# Autodesk Inventor assembly: engine working 1
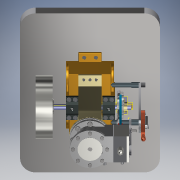
[picture p0: Inventor's stored thumbnail of the model, 180x180]
Saved by Autodesk Inventor 2017 (Build 210142000, 142)
## iProperties
Created: 2018-11-18
Part Number: engine working 1
Document SubType Name: Assembly
Designer: User
Author: User
## Documents named in this file (45)
- E:\Sahil's engine\engine working 1.iam
- E:\Sahil's engine\reverse gear base cast 2.ipt
- E:\Sahil's engine\reverse gear fly wheel.ipt
- E:\Sahil's engine\reverse gear crankshaft outer rod.ipt
- E:\Sahil's engine\reverse gear crankshaft counter weight 2.ipt
- E:\Sahil's engine\reverse gear crankshaft center rod.ipt
- E:\Sahil's engine\reverse gear  upper base bearing holder 1.ipt
- E:\Sahil's engine\reverse gear lower base bearing holder.ipt
- E:\Sahil's engine\reverse gear connecting rod 1.ipt
- E:\Sahil's engine\reverse gear bearing keeper.ipt
- E:\Sahil's engine\reverse gear crank rod 1.ipt
- E:\Sahil's engine\reverse gear crankrod pin 1.ipt
- E:\Sahil's engine\reverse gear cross head 1.ipt
- E:\Sahil's engine\reverse gear pistion rod.ipt
- E:\Sahil's engine\reverse gear piston.ipt
- E:\Sahil's engine\reverse gear stand.ipt
- C:\Users\User\Documents\Inventor\Content Center Files\R2017\en-US\AS 1427(03)\AS 1427 - M3 x 6(1).ipt
- E:\Sahil's engine\reverse gear standard 101.ipt
- E:\Sahil's engine\reverse gear lower cylinder cover.ipt
- E:\Sahil's engine\reverse gear cylinder.ipt
- E:\Sahil's engine\valvle plate.ipt
- E:\Sahil's engine\reverse gear steam chest.ipt
- E:\Sahil's engine\reverse gear steam chest cover.ipt
- E:\Sahil's engine\reverse gear lever ring stud.ipt
- E:\Sahil's engine\reverse gear eccentric 1.ipt
- E:\Sahil's engine\reverse gear lower trap.ipt
- E:\Sahil's engine\reverse gear trap holders.ipt
- E:\Sahil's engine\reverse gear essentric rod 2.ipt
- E:\Sahil's engine\reverse gear reverse lever ring.ipt
- E:\Sahil's engine\reverse gear blands.ipt
- E:\Sahil's engine\reverse gear steam chest rod valve 1.ipt
- E:\Sahil's engine\reverse gear steam chest side valve.ipt
- E:\Sahil's engine\reverse gear gear link.ipt
- E:\Sahil's engine\reverse gear rever lever.ipt
- E:\Sahil's engine\reverse gear link lever 1.ipt
- E:\Sahil's engine\reverse gear drag link.ipt
- E:\Sahil's engine\reverse gear reverse gear.ipt
- E:\Sahil's engine\reverse gear link block.ipt
- E:\Sahil's engine\AS 1427 - M2.5 x 5(1).ipt
- E:\Sahil's engine\AS 1421 - M3x5 Cone Point.ipt
- E:\Sahil's engine\AS 1427 - M3.5 x 6(1).ipt
- E:\Sahil's engine\reverse gear cylinder piping connector 2.ipt
- E:\Sahil's engine\DIN 84 - M3 x 4.ipt
- E:\Sahil's engine\DIN 84 - M4 x 14.ipt
- E:\Sahil's engine\reverse gear link rod.ipt
## Components (94 placed, 44 different names)
1. reverse gear fly wheel:1 — Insert:6, Mate:2, Mate:6, Rotation:3
2. reverse gear crankshaft outer rod:1 — Insert:6, Mate:2, Mate:3, Insert:7, Mate:6, Rotation:1, Mate:51
3. reverse gear crankshaft counter weight 2:2 — Insert:4, Insert:5, Mate:41, Rotation:3
4. reverse gear crankshaft center rod:1 — Insert:4, Insert:8, Rotation:1, Mate:50
5. reverse gear crankshaft outer rod:2 — Insert:5, Mate:3, Insert:22, Insert:23, Mate:41, Mate:120
6. reverse gear  upper base bearing holder 1:1 — Mate:4, Flush:1, Flush:2, Flush:3, Flush:4, Mate:84, Flush:38, Mate:90, Mate:91, Mate:92, Mate:93, Flush:44, Flush:45, Flush:46, Flush:47
7. reverse gear lower base bearing holder:1 — Mate:4, Flush:1, Flush:2, Insert:7, Mate:5
8. reverse gear base cast 2:1 — Mate:5, Flush:3, Flush:4, Mate:9, Flush:7, Flush:8, Flush:15, Flush:16, Mate:13, Insert:13, Insert:14, Insert:15, Insert:16, Mate:14, Flush:17, Flush:18, Insert:20, Insert:21, Mate:53
9. reverse gear  upper base bearing holder 1:2 — Mate:8, Flush:5, Flush:6, Flush:8, Mate:85, Flush:39, Mate:86, Mate:87, Mate:88, Mate:89, Flush:40, Flush:41, Flush:42, Flush:43
10. reverse gear lower base bearing holder:2 — Mate:8, Flush:5, Flush:6, Mate:9, Flush:7
11. reverse gear connecting rod 1:1 — Mate:10, Flush:9, Flush:10, Insert:8, Mate:45, Mate:46, Mate:47, Mate:52
12. reverse gear connecting rod 1:2 — Mate:10, Flush:9, Flush:10, Mate:11, Flush:11, Flush:12
13. reverse gear bearing keeper:1 — Mate:11, Flush:11, Flush:12
14. reverse gear crankrod pin 1:1 — Mate:61, Mate:62
15. reverse gear cross head 1:1 — Mate:57, Mate:59, Mate:60
16. reverse gear pistion rod:1 — Mate:54, Mate:55, Mate:56, Mate:57
17. reverse gear piston:1 — Angle:2, Mate:54, Mate:55, Flush:30
18. reverse gear stand:1 — Flush:15, Flush:16, Mate:13, Angle:1, Angle:2
19. AS 1427 - Metric M3 x 6:1 — Insert:14
20. AS 1427 - Metric M3 x 6:2 — Insert:16
21. AS 1427 - Metric M3 x 6:3 — Insert:15
22. AS 1427 - Metric M3 x 6:4 — Insert:13
23. reverse gear standard 101:1 — Mate:14, Flush:17, Flush:18, Insert:18, Mate:56, Flush:32, Mate:78, Mate:79, Flush:33, Mate:80, Flush:34, Mate:81, Flush:35, Mate:82, Flush:36, Mate:83, Flush:37
24. reverse gear lower cylinder cover:1 — Insert:18, Insert:19, Mate:32, Mate:33, Mate:34
25. reverse gear cylinder:1 — Insert:19, Mate:15, Flush:19, Flush:20, Flush:21, Flush:22, Mate:32, Mate:33, Mate:34, Insert:30, Mate:102, Flush:56, Mate:103, Flush:57, Mate:104, Flush:58, Mate:105, Flush:59, Mate:106, Flush:60, Mate:107, Flush:61, Mate:108, Flush:62, Mate:109, Flush:63, Mate:110, Flush:64, Mate:111, Flush:65, Mate:112, Flush:66, Mate:113, Flush:67, Mate:114, Flush:68
26. valvle plate:1 — Mate:15, Flush:19, Flush:20, Mate:16
27. reverse gear steam chest:1 — Mate:16, Flush:21, Flush:22, Mate:17, Flush:23, Flush:24, Insert:29, Mate:69, Mate:70, Insert:31, Mate:124
28. reverse gear steam chest cover:1 — Mate:17, Flush:23, Flush:24, Angle:1, Mate:63, Mate:64, Mate:65, Mate:94, Flush:48, Mate:95, Flush:49, Mate:96, Flush:50, Mate:97, Flush:51, Mate:98, Flush:52, Mate:99, Flush:53, Mate:100, Flush:54, Mate:101, Flush:55
29. reverse gear lever ring stud:1 — Insert:20, Mate:39
30. reverse gear lever ring stud:2 — Insert:21, Mate:29
31. reverse gear eccentric 1:1 — Insert:22, Insert:24
32. reverse gear eccentric 1:2 — Insert:23, Insert:25, Mate:120
33. reverse gear lower trap:1 — Mate:20, Mate:21, Flush:26
34. reverse gear lower trap:2 — Mate:18, Mate:19, Flush:25
35. reverse gear trap holders:1 — Insert:24, Mate:18, Mate:19, Flush:25, Insert:27
36. reverse gear trap holders:2 — Insert:25, Mate:20, Mate:21, Flush:26, Insert:26
37. reverse gear essentric rod 2:1 — Insert:27, Mate:76
38. reverse gear essentric rod 2:2 — Insert:26, Mate:77
39. reverse gear reverse lever ring:1 — Mate:29, Mate:39, Mate:67, Mate:68
40. reverse gear blands:1 — Insert:29
41. reverse gear steam chest rod valve 1:1 — Mate:70, Mate:71, Mate:72, Mate:73, Mate:122
42. reverse gear steam chest side valve:1 — Mate:69, Mate:71, Mate:72, Mate:124
43. reverse gear gear link:1 — Mate:63, Mate:64, Mate:65
44. reverse gear link lever 1:1 — Mate:125, Mate:126, Mate:128, Flush:71
45. reverse gear drag link:1 — Mate:115, Mate:116, Mate:118
46. reverse gear crank rod 1:1 — Mate:45, Mate:46, Mate:47, Mate:59, Mate:61, Mate:62
47. reverse gear crankshaft counter weight 2:3 — Mate:50, Mate:51, Mate:52, Mate:53
48. reverse gear rever lever:2 — Mate:67, Mate:68, Mate:115, Mate:116, Mate:125, Mate:126, Mate:127, Flush:70, Mate:129, Flush:72
49. reverse gear reverse gear:1 — Mate:73, Mate:76, Mate:77, Mate:117, Mate:119, Mate:121, Flush:69, Mate:123
50. AS 1427 - Metric M2.5 x 5:1 — Flush:32, Mate:78, Rotation:4
51. AS 1427 - Metric M2.5 x 5:2 — Mate:83, Flush:37, Rotation:7
52. AS 1427 - Metric M2.5 x 5:3 — Mate:82, Flush:36, Rotation:6, Rotation:7
53. AS 1427 - Metric M2.5 x 5:4 — Mate:80, Flush:34, Rotation:5
54. AS 1427 - Metric M2.5 x 5:5 — Mate:79, Flush:33, Rotation:4, Rotation:5
55. AS 1427 - Metric M2.5 x 5:6 — Mate:81, Flush:35, Rotation:6
56. AS 1421 Cone Point - Metric M3x5 Cone Point:1 — Mate:85, Flush:39
57. AS 1421 Cone Point - Metric M3x5 Cone Point:2 — Mate:84, Flush:38
58. AS 1427 - Metric M3.5 x 6:1 — Mate:89, Flush:43
59. AS 1427 - Metric M3.5 x 6:2 — Mate:87, Flush:41
60. AS 1427 - Metric M3.5 x 6:3 — Mate:88, Flush:42
61. AS 1427 - Metric M3.5 x 6:4 — Mate:86, Flush:40
62. AS 1427 - Metric M3.5 x 6:5 — Mate:92, Flush:46
63. AS 1427 - Metric M3.5 x 6:6 — Mate:93, Flush:47
64. AS 1427 - Metric M3.5 x 6:7 — Mate:90, Flush:44
65. AS 1427 - Metric M3.5 x 6:8 — Mate:91, Flush:45
66. reverse gear cylinder piping connector 2:1 — Insert:31
67. reverse gear cylinder piping connector 2:2 — Insert:30
68. AS 1427 - Metric M3.5 x 6:9 — Mate:98, Flush:52
69. AS 1427 - Metric M3.5 x 6:10 — Mate:97, Flush:51
70. AS 1427 - Metric M3.5 x 6:11 — Mate:99, Flush:53
71. AS 1427 - Metric M3.5 x 6:12 — Mate:101, Flush:55
72. AS 1427 - Metric M3.5 x 6:13 — Mate:100, Flush:54
73. AS 1427 - Metric M3.5 x 6:14 — Mate:94, Flush:48
74. AS 1427 - Metric M3.5 x 6:15 — Mate:95, Flush:49
75. AS 1427 - Metric M3.5 x 6:16 — Mate:96, Flush:50
76. DIN 84 - replaced by DIN EN ISO 1207 M3 x 4:1 — Mate:104, Flush:58
77. DIN 84 - replaced by DIN EN ISO 1207 M3 x 4:2 — Mate:103, Flush:57
78. DIN 84 - replaced by DIN EN ISO 1207 M3 x 4:3 — Mate:106, Flush:60
79. DIN 84 - replaced by DIN EN ISO 1207 M3 x 4:4 — Mate:105, Flush:59
80. DIN 84 - replaced by DIN EN ISO 1207 M3 x 4:5 — Mate:107, Flush:61
81. DIN 84 - replaced by DIN EN ISO 1207 M3 x 4:6 — Mate:108, Flush:62
82. DIN 84 - replaced by DIN EN ISO 1207 M3 x 4:7 — Mate:109, Flush:63
83. DIN 84 - replaced by DIN EN ISO 1207 M3 x 4:8 — Mate:102, Flush:56
84. DIN 84 - replaced by DIN EN ISO 1207 M4 x 14:7 — Mate:110, Flush:64
85. DIN 84 - replaced by DIN EN ISO 1207 M4 x 14:8 — Mate:112, Flush:66
86. DIN 84 - replaced by DIN EN ISO 1207 M4 x 14:9 — Mate:111, Flush:65
87. DIN 84 - replaced by DIN EN ISO 1207 M4 x 14:11 — Mate:114, Flush:68
88. DIN 84 - replaced by DIN EN ISO 1207 M4 x 14:12 — Mate:113, Flush:67
89. reverse gear link rod:1 — Mate:117, Mate:118, Mate:119
90. reverse gear link block:1 — Mate:121
91. reverse gear link block:2 — Mate:122, Flush:69, Mate:123
92. AS 1427 - Metric M3.5 x 6:17 — Mate:127, Flush:70
93. AS 1427 - Metric M3.5 x 6:18 — Mate:128, Flush:71
94. AS 1427 - Metric M3.5 x 6:19 — Mate:129, Flush:72
## Relationships (199: Mate 103, Flush 66, Insert 22, RelateRotation 6, Angle 2)
- Insert:4: reverse gear crankshaft counter weight 2:2 ↔ reverse gear crankshaft center rod:1
- Insert:5 (-4 mm): reverse gear crankshaft counter weight 2:2 ↔ reverse gear crankshaft outer rod:2
- Insert:6 (-5 mm): reverse gear fly wheel:1 ↔ reverse gear crankshaft outer rod:1
- Mate:2: reverse gear fly wheel:1 ↔ reverse gear crankshaft outer rod:1
- Mate:3: reverse gear crankshaft outer rod:1 ↔ reverse gear crankshaft outer rod:2
- Mate:4: reverse gear  upper base bearing holder 1:1 ↔ reverse gear lower base bearing holder:1
- Flush:1: reverse gear  upper base bearing holder 1:1 ↔ reverse gear lower base bearing holder:1
- Flush:2 (7 mm): reverse gear  upper base bearing holder 1:1 ↔ reverse gear lower base bearing holder:1
- Insert:7 (-15 mm): reverse gear crankshaft outer rod:1 ↔ reverse gear lower base bearing holder:1
- Mate:5: reverse gear lower base bearing holder:1 ↔ reverse gear base cast 2:1
- Flush:3 (29 mm): reverse gear  upper base bearing holder 1:1 ↔ reverse gear base cast 2:1
- Flush:4: reverse gear  upper base bearing holder 1:1 ↔ reverse gear base cast 2:1
- Mate:6: reverse gear fly wheel:1 ↔ reverse gear crankshaft outer rod:1
- Mate:8: reverse gear  upper base bearing holder 1:2 ↔ reverse gear lower base bearing holder:2
- Flush:5 (7 mm): reverse gear  upper base bearing holder 1:2 ↔ reverse gear lower base bearing holder:2
- Flush:6: reverse gear  upper base bearing holder 1:2 ↔ reverse gear lower base bearing holder:2
- Mate:9: reverse gear base cast 2:1 ↔ reverse gear lower base bearing holder:2
- Flush:7: reverse gear base cast 2:1 ↔ reverse gear lower base bearing holder:2
- Flush:8 (29 mm): reverse gear base cast 2:1 ↔ reverse gear  upper base bearing holder 1:2
- Mate:10: reverse gear connecting rod 1:1 ↔ reverse gear connecting rod 1:2
- Flush:9: reverse gear connecting rod 1:1 ↔ reverse gear connecting rod 1:2
- Flush:10: reverse gear connecting rod 1:1 ↔ reverse gear connecting rod 1:2
- Mate:11: reverse gear connecting rod 1:2 ↔ reverse gear bearing keeper:1
- Flush:11: reverse gear connecting rod 1:2 ↔ reverse gear bearing keeper:1
- Flush:12: reverse gear connecting rod 1:2 ↔ reverse gear bearing keeper:1
- Insert:8 (5.5 mm): reverse gear crankshaft center rod:1 ↔ reverse gear connecting rod 1:1
- Flush:15 (-58 mm): reverse gear base cast 2:1 ↔ reverse gear stand:1
- Flush:16 (53 mm): reverse gear base cast 2:1 ↔ reverse gear stand:1
- Mate:13: reverse gear base cast 2:1 ↔ reverse gear stand:1
- Insert:13 (-5.5 mm): reverse gear base cast 2:1 ↔ AS 1427 - Metric M3 x 6:4
- Insert:14 (-5.5 mm): reverse gear base cast 2:1 ↔ AS 1427 - Metric M3 x 6:1
- Insert:15 (-5.5 mm): reverse gear base cast 2:1 ↔ AS 1427 - Metric M3 x 6:3
- Insert:16 (-5.5 mm): reverse gear base cast 2:1 ↔ AS 1427 - Metric M3 x 6:2
- Mate:14: reverse gear base cast 2:1 ↔ reverse gear standard 101:1
- Flush:17: reverse gear base cast 2:1 ↔ reverse gear standard 101:1
- Flush:18 (12 mm): reverse gear base cast 2:1 ↔ reverse gear standard 101:1
- Insert:18 (-6.5 mm): reverse gear standard 101:1 ↔ reverse gear lower cylinder cover:1
- Insert:19: reverse gear lower cylinder cover:1 ↔ reverse gear cylinder:1
- Mate:15: reverse gear cylinder:1 ↔ valvle plate:1
- Flush:19: reverse gear cylinder:1 ↔ valvle plate:1
- Flush:20: reverse gear cylinder:1 ↔ valvle plate:1
- Mate:16: valvle plate:1 ↔ reverse gear steam chest:1
- Flush:21: reverse gear cylinder:1 ↔ reverse gear steam chest:1
- Flush:22: reverse gear cylinder:1 ↔ reverse gear steam chest:1
- Mate:17: reverse gear steam chest:1 ↔ reverse gear steam chest cover:1
- Flush:23: reverse gear steam chest:1 ↔ reverse gear steam chest cover:1
- Flush:24: reverse gear steam chest:1 ↔ reverse gear steam chest cover:1
- Insert:20 (-4.8 mm): reverse gear base cast 2:1 ↔ reverse gear lever ring stud:1
- Insert:21 (-4.8 mm): reverse gear base cast 2:1 ↔ reverse gear lever ring stud:2
- Insert:22 (-18 mm): reverse gear crankshaft outer rod:2 ↔ reverse gear eccentric 1:1
- Insert:23 (-14 mm): reverse gear crankshaft outer rod:2 ↔ reverse gear eccentric 1:2
- Insert:24: reverse gear eccentric 1:1 ↔ reverse gear trap holders:1
- Mate:18: reverse gear lower trap:2 ↔ reverse gear trap holders:1
- Mate:19: reverse gear lower trap:2 ↔ reverse gear trap holders:1
- Flush:25: reverse gear lower trap:2 ↔ reverse gear trap holders:1
- Insert:25: reverse gear eccentric 1:2 ↔ reverse gear trap holders:2
- Mate:20: reverse gear lower trap:1 ↔ reverse gear trap holders:2
- Mate:21: reverse gear lower trap:1 ↔ reverse gear trap holders:2
- Flush:26: reverse gear lower trap:1 ↔ reverse gear trap holders:2
- Insert:26 (-3.7 mm): reverse gear trap holders:2 ↔ reverse gear essentric rod 2:2
- Insert:27 (-3.7 mm): reverse gear trap holders:1 ↔ reverse gear essentric rod 2:1
- Rotation:1 [RelateRotation] (1 ul): reverse gear crankshaft outer rod:1 ↔ reverse gear crankshaft center rod:1
- Insert:29 (-8 mm): reverse gear steam chest:1 ↔ reverse gear blands:1
- Mate:29: reverse gear lever ring stud:2 ↔ reverse gear reverse lever ring:1
- Mate:32: reverse gear lower cylinder cover:1 ↔ reverse gear cylinder:1
- Mate:33: reverse gear lower cylinder cover:1 ↔ reverse gear cylinder:1
- Mate:34: reverse gear lower cylinder cover:1 ↔ reverse gear cylinder:1
- Angle:1 (0 deg): reverse gear stand:1 ↔ reverse gear steam chest cover:1
- Mate:39: reverse gear lever ring stud:1 ↔ reverse gear reverse lever ring:1
- Mate:41: reverse gear crankshaft counter weight 2:2 ↔ reverse gear crankshaft outer rod:2
- Angle:2 (0 deg): reverse gear piston:1 ↔ reverse gear stand:1
- Mate:45: reverse gear connecting rod 1:1 ↔ reverse gear crank rod 1:1
- Mate:46: reverse gear connecting rod 1:1 ↔ reverse gear crank rod 1:1
- Mate:47: reverse gear connecting rod 1:1 ↔ reverse gear crank rod 1:1
- Mate:50: reverse gear crankshaft center rod:1 ↔ reverse gear crankshaft counter weight 2:3
- Mate:51: reverse gear crankshaft outer rod:1 ↔ reverse gear crankshaft counter weight 2:3
- Mate:52: reverse gear connecting rod 1:1 ↔ reverse gear crankshaft counter weight 2:3
- Mate:53 (2.25 mm): reverse gear base cast 2:1 ↔ reverse gear crankshaft counter weight 2:3
- Mate:54: reverse gear pistion rod:1 ↔ reverse gear piston:1
- Mate:55: reverse gear pistion rod:1 ↔ reverse gear piston:1
- Mate:56: reverse gear pistion rod:1 ↔ reverse gear standard 101:1
- Mate:57: reverse gear cross head 1:1 ↔ reverse gear pistion rod:1
- Mate:59: reverse gear cross head 1:1 ↔ reverse gear crank rod 1:1
- Flush:30 (45 mm): reverse gear piston:1
- Mate:60: reverse gear cross head 1:1
- Mate:61: reverse gear crankrod pin 1:1 ↔ reverse gear crank rod 1:1
- Mate:62: reverse gear crankrod pin 1:1 ↔ reverse gear crank rod 1:1
- Rotation:3 [RelateRotation] (2.05 ul): reverse gear fly wheel:1 ↔ reverse gear crankshaft counter weight 2:2
- Mate:63: reverse gear steam chest cover:1 ↔ reverse gear gear link:1
- Mate:64: reverse gear steam chest cover:1 ↔ reverse gear gear link:1
- Mate:65: reverse gear steam chest cover:1 ↔ reverse gear gear link:1
- Mate:67: reverse gear reverse lever ring:1 ↔ reverse gear rever lever:2
- Mate:68: reverse gear reverse lever ring:1 ↔ reverse gear rever lever:2
- Mate:69: reverse gear steam chest:1 ↔ reverse gear steam chest side valve:1
- Mate:70: reverse gear steam chest:1 ↔ reverse gear steam chest rod valve 1:1
- Mate:71: reverse gear steam chest rod valve 1:1 ↔ reverse gear steam chest side valve:1
- Mate:72: reverse gear steam chest rod valve 1:1 ↔ reverse gear steam chest side valve:1
- Mate:73: reverse gear steam chest rod valve 1:1 ↔ reverse gear reverse gear:1
- Mate:76: reverse gear essentric rod 2:1 ↔ reverse gear reverse gear:1
- Mate:77: reverse gear essentric rod 2:2 ↔ reverse gear reverse gear:1
- Flush:32: reverse gear standard 101:1 ↔ AS 1427 - Metric M2.5 x 5:1
- Mate:78: reverse gear standard 101:1 ↔ AS 1427 - Metric M2.5 x 5:1
- Mate:79: reverse gear standard 101:1 ↔ AS 1427 - Metric M2.5 x 5:5
- Flush:33: reverse gear standard 101:1 ↔ AS 1427 - Metric M2.5 x 5:5
- Mate:80: reverse gear standard 101:1 ↔ AS 1427 - Metric M2.5 x 5:4
- Flush:34: reverse gear standard 101:1 ↔ AS 1427 - Metric M2.5 x 5:4
- Rotation:4 [RelateRotation] (1 ul): AS 1427 - Metric M2.5 x 5:1 ↔ AS 1427 - Metric M2.5 x 5:5
- Rotation:5 [RelateRotation] (1 ul): AS 1427 - Metric M2.5 x 5:4 ↔ AS 1427 - Metric M2.5 x 5:5
- Mate:81: reverse gear standard 101:1 ↔ AS 1427 - Metric M2.5 x 5:6
- Flush:35: reverse gear standard 101:1 ↔ AS 1427 - Metric M2.5 x 5:6
- Mate:82: reverse gear standard 101:1 ↔ AS 1427 - Metric M2.5 x 5:3
- Flush:36: reverse gear standard 101:1 ↔ AS 1427 - Metric M2.5 x 5:3
- Mate:83: reverse gear standard 101:1 ↔ AS 1427 - Metric M2.5 x 5:2
- Flush:37: reverse gear standard 101:1 ↔ AS 1427 - Metric M2.5 x 5:2
- Rotation:6 [RelateRotation] (1 ul): AS 1427 - Metric M2.5 x 5:3 ↔ AS 1427 - Metric M2.5 x 5:6
- Rotation:7 [RelateRotation] (1 ul): AS 1427 - Metric M2.5 x 5:2 ↔ AS 1427 - Metric M2.5 x 5:3
- Mate:84: reverse gear  upper base bearing holder 1:1 ↔ AS 1421 Cone Point - Metric M3x5 Cone Point:2
- Flush:38: reverse gear  upper base bearing holder 1:1 ↔ AS 1421 Cone Point - Metric M3x5 Cone Point:2
- Mate:85: reverse gear  upper base bearing holder 1:2 ↔ AS 1421 Cone Point - Metric M3x5 Cone Point:1
- Flush:39: reverse gear  upper base bearing holder 1:2 ↔ AS 1421 Cone Point - Metric M3x5 Cone Point:1
- Mate:86: reverse gear  upper base bearing holder 1:2 ↔ AS 1427 - Metric M3.5 x 6:4
- Mate:87: reverse gear  upper base bearing holder 1:2 ↔ AS 1427 - Metric M3.5 x 6:2
- Mate:88: reverse gear  upper base bearing holder 1:2 ↔ AS 1427 - Metric M3.5 x 6:3
- Mate:89: reverse gear  upper base bearing holder 1:2 ↔ AS 1427 - Metric M3.5 x 6:1
- Flush:40 (-1 mm): reverse gear  upper base bearing holder 1:2 ↔ AS 1427 - Metric M3.5 x 6:4
- Flush:41 (1 mm): reverse gear  upper base bearing holder 1:2 ↔ AS 1427 - Metric M3.5 x 6:2
- Flush:42 (-1 mm): reverse gear  upper base bearing holder 1:2 ↔ AS 1427 - Metric M3.5 x 6:3
- Flush:43 (-1 mm): reverse gear  upper base bearing holder 1:2 ↔ AS 1427 - Metric M3.5 x 6:1
- Mate:90: reverse gear  upper base bearing holder 1:1 ↔ AS 1427 - Metric M3.5 x 6:7
- Mate:91: reverse gear  upper base bearing holder 1:1 ↔ AS 1427 - Metric M3.5 x 6:8
- Mate:92: reverse gear  upper base bearing holder 1:1 ↔ AS 1427 - Metric M3.5 x 6:5
- Mate:93: reverse gear  upper base bearing holder 1:1 ↔ AS 1427 - Metric M3.5 x 6:6
- Flush:44 (1 mm): reverse gear  upper base bearing holder 1:1 ↔ AS 1427 - Metric M3.5 x 6:7
- Flush:45 (1 mm): reverse gear  upper base bearing holder 1:1 ↔ AS 1427 - Metric M3.5 x 6:8
- Flush:46 (-1 mm): reverse gear  upper base bearing holder 1:1 ↔ AS 1427 - Metric M3.5 x 6:5
- Flush:47 (-1 mm): reverse gear  upper base bearing holder 1:1 ↔ AS 1427 - Metric M3.5 x 6:6
- Insert:30: reverse gear cylinder:1 ↔ reverse gear cylinder piping connector 2:2
- Insert:31 (-4 mm): reverse gear steam chest:1 ↔ reverse gear cylinder piping connector 2:1
- Mate:94: reverse gear steam chest cover:1 ↔ AS 1427 - Metric M3.5 x 6:14
- Flush:48 (-0.5 mm): reverse gear steam chest cover:1 ↔ AS 1427 - Metric M3.5 x 6:14
- Mate:95: reverse gear steam chest cover:1 ↔ AS 1427 - Metric M3.5 x 6:15
- Flush:49 (-0.5 mm): reverse gear steam chest cover:1 ↔ AS 1427 - Metric M3.5 x 6:15
- Mate:96: reverse gear steam chest cover:1 ↔ AS 1427 - Metric M3.5 x 6:16
- Flush:50 (-0.5 mm): reverse gear steam chest cover:1 ↔ AS 1427 - Metric M3.5 x 6:16
- Mate:97: reverse gear steam chest cover:1 ↔ AS 1427 - Metric M3.5 x 6:10
- Flush:51 (-0.5 mm): reverse gear steam chest cover:1 ↔ AS 1427 - Metric M3.5 x 6:10
- Mate:98: reverse gear steam chest cover:1 ↔ AS 1427 - Metric M3.5 x 6:9
- Flush:52 (-0.5 mm): reverse gear steam chest cover:1 ↔ AS 1427 - Metric M3.5 x 6:9
- Mate:99: reverse gear steam chest cover:1 ↔ AS 1427 - Metric M3.5 x 6:11
- Flush:53 (-0.5 mm): reverse gear steam chest cover:1 ↔ AS 1427 - Metric M3.5 x 6:11
- Mate:100: reverse gear steam chest cover:1 ↔ AS 1427 - Metric M3.5 x 6:13
- Flush:54 (-0.5 mm): reverse gear steam chest cover:1 ↔ AS 1427 - Metric M3.5 x 6:13
- Mate:101: reverse gear steam chest cover:1 ↔ AS 1427 - Metric M3.5 x 6:12
- Flush:55 (-0.5 mm): reverse gear steam chest cover:1 ↔ AS 1427 - Metric M3.5 x 6:12
- Mate:102: reverse gear cylinder:1 ↔ DIN 84 - replaced by DIN EN ISO 1207 M3 x 4:8
- Flush:56 (-2.5 mm): reverse gear cylinder:1 ↔ DIN 84 - replaced by DIN EN ISO 1207 M3 x 4:8
- Mate:103: reverse gear cylinder:1 ↔ DIN 84 - replaced by DIN EN ISO 1207 M3 x 4:2
- Flush:57 (-2.5 mm): reverse gear cylinder:1 ↔ DIN 84 - replaced by DIN EN ISO 1207 M3 x 4:2
- Mate:104: reverse gear cylinder:1 ↔ DIN 84 - replaced by DIN EN ISO 1207 M3 x 4:1
- Flush:58 (-2.5 mm): reverse gear cylinder:1 ↔ DIN 84 - replaced by DIN EN ISO 1207 M3 x 4:1
- Mate:105: reverse gear cylinder:1 ↔ DIN 84 - replaced by DIN EN ISO 1207 M3 x 4:4
- Flush:59 (-2.5 mm): reverse gear cylinder:1 ↔ DIN 84 - replaced by DIN EN ISO 1207 M3 x 4:4
- Mate:106: reverse gear cylinder:1 ↔ DIN 84 - replaced by DIN EN ISO 1207 M3 x 4:3
- Flush:60 (-2.5 mm): reverse gear cylinder:1 ↔ DIN 84 - replaced by DIN EN ISO 1207 M3 x 4:3
- Mate:107: reverse gear cylinder:1 ↔ DIN 84 - replaced by DIN EN ISO 1207 M3 x 4:5
- Flush:61 (-2.5 mm): reverse gear cylinder:1 ↔ DIN 84 - replaced by DIN EN ISO 1207 M3 x 4:5
- Mate:108: reverse gear cylinder:1 ↔ DIN 84 - replaced by DIN EN ISO 1207 M3 x 4:6
- Flush:62 (-2.5 mm): reverse gear cylinder:1 ↔ DIN 84 - replaced by DIN EN ISO 1207 M3 x 4:6
- Mate:109: reverse gear cylinder:1 ↔ DIN 84 - replaced by DIN EN ISO 1207 M3 x 4:7
- Flush:63 (-2.5 mm): reverse gear cylinder:1 ↔ DIN 84 - replaced by DIN EN ISO 1207 M3 x 4:7
- Mate:110: reverse gear cylinder:1 ↔ DIN 84 - replaced by DIN EN ISO 1207 M4 x 14:7
- Flush:64 (-4 mm): reverse gear cylinder:1 ↔ DIN 84 - replaced by DIN EN ISO 1207 M4 x 14:7
- Mate:111: reverse gear cylinder:1 ↔ DIN 84 - replaced by DIN EN ISO 1207 M4 x 14:9
- Flush:65 (-4 mm): reverse gear cylinder:1 ↔ DIN 84 - replaced by DIN EN ISO 1207 M4 x 14:9
- Mate:112: reverse gear cylinder:1 ↔ DIN 84 - replaced by DIN EN ISO 1207 M4 x 14:8
- Flush:66 (-4 mm): reverse gear cylinder:1 ↔ DIN 84 - replaced by DIN EN ISO 1207 M4 x 14:8
- Mate:113: reverse gear cylinder:1 ↔ DIN 84 - replaced by DIN EN ISO 1207 M4 x 14:12
- Flush:67 (-4 mm): reverse gear cylinder:1 ↔ DIN 84 - replaced by DIN EN ISO 1207 M4 x 14:12
- Mate:114: reverse gear cylinder:1 ↔ DIN 84 - replaced by DIN EN ISO 1207 M4 x 14:11
- Flush:68 (-4 mm): reverse gear cylinder:1 ↔ DIN 84 - replaced by DIN EN ISO 1207 M4 x 14:11
- Mate:115: reverse gear drag link:1 ↔ reverse gear rever lever:2
- Mate:116: reverse gear drag link:1 ↔ reverse gear rever lever:2
- Mate:117: reverse gear reverse gear:1 ↔ reverse gear link rod:1
- Mate:118: reverse gear drag link:1 ↔ reverse gear link rod:1
- Mate:119: reverse gear reverse gear:1 ↔ reverse gear link rod:1
- Mate:120: reverse gear crankshaft outer rod:2 ↔ reverse gear eccentric 1:2
- Mate:121: reverse gear reverse gear:1 ↔ reverse gear link block:1
- Mate:122: reverse gear steam chest rod valve 1:1 ↔ reverse gear link block:2
- Flush:69: reverse gear reverse gear:1 ↔ reverse gear link block:2
- Mate:123 (-4 mm): reverse gear reverse gear:1 ↔ reverse gear link block:2
- Mate:124: reverse gear steam chest:1 ↔ reverse gear steam chest side valve:1
- Mate:125: reverse gear link lever 1:1 ↔ reverse gear rever lever:2
- Mate:126: reverse gear link lever 1:1 ↔ reverse gear rever lever:2
- Mate:127: reverse gear rever lever:2 ↔ AS 1427 - Metric M3.5 x 6:17
- Flush:70 (-1 mm): reverse gear rever lever:2 ↔ AS 1427 - Metric M3.5 x 6:17
- Mate:128: reverse gear link lever 1:1 ↔ AS 1427 - Metric M3.5 x 6:18
- Flush:71 (-1 mm): reverse gear link lever 1:1 ↔ AS 1427 - Metric M3.5 x 6:18
- Mate:129: reverse gear rever lever:2 ↔ AS 1427 - Metric M3.5 x 6:19
- Flush:72 (-1 mm): reverse gear rever lever:2 ↔ AS 1427 - Metric M3.5 x 6:19
